# Autodesk Inventor assembly: Tred_Assembly2
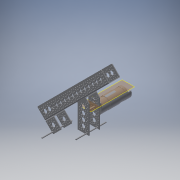
[picture p0: Inventor's stored thumbnail of the model, 180x180]
Saved by Autodesk Inventor 2016 (Build 200138000, 138)
## iProperties
Created: 2015-10-03
Part Number: Tred_Assembly2
Document SubType Name: Assembly
Designer: steve.brooks
Author: steve.brooks
## Documents named in this file (7)
- C:\Robotics\2015-16_CAD\Tred_Assembly2.iam
- C:\Users\steve.brooks\Documents\COTSParts\Motors\Andymark 2964  NeveRest 40 Motor.ipt
- C:\Users\steve.brooks\Documents\COTSParts\All STEP Files\555 parts\555128.ipt
- C:\Users\steve.brooks\Documents\COTSParts\All STEP Files\585 parts\585482.ipt
- C:\Robotics\2015-16_CAD\COTSParts\Actobotics\585 parts\585454.ipt
- C:\Robotics\2015-16_CAD\COTSParts\Actobotics\585 parts\585440.ipt
- C:\Robotics\2015-16_CAD\custom cad parts\4 in x .140 in rod.ipt
## Components (7 placed, 6 different names)
1. Andymark 2964  NeveRest 40 Motor:1 — Mate:1, Angle:1, Tangent:1, Tangent:2
2. 555128:1 — Mate:1, Flush:1, Tangent:2, Mate:2, Mate:3, Mate:4
3. 585482:1 — Mate:2, Mate:3, Mate:4, Mate:5, Mate:6, Mate:7, Mate:11, Mate:12, Flush:2
4. 585454:1 — Mate:5, Mate:6, Mate:7, Mate:8, Mate:9, Mate:10
5. 585440:1 — Mate:8, Mate:9, Mate:10, Mate:13, Mate:14, Flush:3
6. 4 in x .140 in rod:1 — Mate:11, Mate:12, Flush:2
7. 4 in x .140 in rod:2 — Mate:13, Mate:14, Flush:3
## Relationships (20: Mate 14, Flush 3, Tangent 2, Angle 1)
- Mate:1: Andymark 2964  NeveRest 40 Motor:1 ↔ 555128:1
- Angle:1 (0 deg): Andymark 2964  NeveRest 40 Motor:1
- Tangent:1: Andymark 2964  NeveRest 40 Motor:1
- Flush:1 (5.08 mm): 555128:1
- Tangent:2: Andymark 2964  NeveRest 40 Motor:1 ↔ 555128:1
- Mate:2: 555128:1 ↔ 585482:1
- Mate:3: 555128:1 ↔ 585482:1
- Mate:4: 555128:1 ↔ 585482:1
- Mate:5: 585482:1 ↔ 585454:1
- Mate:6: 585482:1 ↔ 585454:1
- Mate:7: 585482:1 ↔ 585454:1
- Mate:8: 585454:1 ↔ 585440:1
- Mate:9: 585454:1 ↔ 585440:1
- Mate:10: 585454:1 ↔ 585440:1
- Mate:11: 585482:1 ↔ 4 in x .140 in rod:1
- Mate:12: 585482:1 ↔ 4 in x .140 in rod:1
- Flush:2 (25.4 mm): 585482:1 ↔ 4 in x .140 in rod:1
- Mate:13: 585440:1 ↔ 4 in x .140 in rod:2
- Mate:14: 585440:1 ↔ 4 in x .140 in rod:2
- Flush:3 (25.4 mm): 585440:1 ↔ 4 in x .140 in rod:2
